# Autodesk Inventor assembly: 021-DXP(F,D-770)
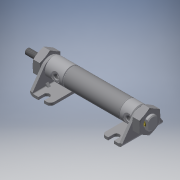
[picture p0: Inventor's stored thumbnail of the model, 180x180]
Saved by Autodesk Inventor 2018 (Build 220112000, 112)
## iProperties
Category: PARTsolutions
Company: BIMBA
Created: 2019-01-18
Part Number: 021-DXP(F,D-770)
Catalog Web Link: www.cadenas.de
Description: Original Line Standard Air Cylinders-Standard Air Cylinders
Vendor: BIMBA
Document SubType Name: Assembly
Designer: psadmin
Manufacturer: BIMBA
PSOL_IDENT_0: {$CADENAS_DATA\23d-libs\bimba\bimba\bimba_imperial\bimba_full_line\original_line_cylinders\standard_
PSOL_IDENT_1: air_cylinders\standard_air_cylinder_asmtab.prj},331 {VTYP=3D},{STYP=ASSTAB},{NB=021-DXP(F,D-770)},{L
PSOL_IDENT_2: INA=021-DXP},{NN=Original Line Standard Air Cylinders},{DATE=21.03.2018 14:31:21},{GEOMDATE=19.03.20
PSOL_IDENT_3: 18 11:39:15},{VERSION=},{LINEID=40},{WBVAR=STROKE,ACTING,MNT,DER,NR,BM,CO,OO,VO,M,EE,EEL,K,Q,Y,G,T,H
PSOL_IDENT_4: L,B,H,SER,SR,NT,W,STPT1,STPT2,STPT3,STPT4,MB,PB,PRC,TB,MN},{WBNUMERIC=STROKE,EEL}  {NB=021-DXP(F,D-7
PSOL_IDENT_5: 70)},{LINA=021-DXP},{KT=DUMMY},{PN=021-DXP},{PNC=021-DXP(F,D-770)},{PNA=(D-770)},{DASH=-},{BORE1=0.5
PSOL_IDENT_6: 6250000},{BORE=9/16\" (02)},{BOREPN=02},{STROKE=1.000},{STROKEALG=[0.011:50/0.001]},{STROKE1=1.000},
PSOL_IDENT_7: {ACTING=D},{ACTINGALG= '' , 'Single Acting (SA)' , 'R' , 'Reverse Single Acting (SA)' , 'D' , 'Doubl
PSOL_IDENT_8: e Acting (SA)' },{ACTINGPN=D},{MNT=XP},{MNTALG= '' , 'Front Nose Mounting (SA)' , 'XP' , 'Double End
PSOL_IDENT_9: or Rear Pivot Mounting (SA)' , 'X' , 'Double End Mounting (SA)' },{TYPE=},{MNTPN=XP},{DER=},{DERALG=
PSOL_IDENT_10: '' , 'N/A' },{NR=},{NRALG= '' , 'N/A' },{NRPN=},{BM=},{BMALG= '' , 'N/A' },{BMPN=},{CO=},{COALG= ''
PSOL_IDENT_11: , 'N/A' },{OO=},{OOALG= '', 'N/A' },{OOPN=},{VO=Z},{VOALG= 'Z' , 'N/A' },{VOPN=},{OOVOPN=},{M=},{MA
PSOL_IDENT_12: LG= '', 'Without Magnet', 'M', 'With Magnet' },{EE=},{EEL=0.000},{EEMAX=49.0000},{EEALG= '', 'Withou
PSOL_IDENT_13: t Extra Extension', 'EE', 'With Extra Extension' },{EELALG=0},{EEPN=},{EEPN1=0.000},{K=},{KALG= '', '
PSOL_IDENT_14: Standard' , 'K' , 'Ports Rotated 90deg K' },{KPN=},{Q=},{QALG= '' , 'N/A' },{QPN=},{Y=},{YALG= '' , '
PSOL_IDENT_15: With Pivot Bushing' },{YPN=},{YCON=Y},{F=},{FALG= '', 'Non-Coated (Standard)', 'F', 'Molycoated' },{
PSOL_IDENT_16: FPN=},{G=},{GPN=},{GPN99=},{T=},{TALG= '' , 'Standard -20° to 200°F (-29° to 95°C)' , 'N' , 'Low Tem
PSOL_IDENT_17: perature' , 'V' , 'High Temperature' },{NPN=},{VPN=},{HL=},{HLALG= '' , 'Without Low Pressure Hydrau
PSOL_IDENT_18: lic' , 'HL' , 'With Low Pressure Hydraulic' },{B=},{BALG= '', 'W/out Bumpers' , 'B' , 'W/ Bumpers' }
PSOL_IDENT_19: ,{BPN=},{H=},{HALG= '', 'N/A' },{HPN=},{SER=},{SERALG= '' , 'Without Spring Extend/Return' , 'JS' , '
PSOL_IDENT_20: With Spring Return' , 'JR' , 'With Spring Extend' },{SR=},{SRALG= '' , 'Standard Stainless Steel' },
PSOL_IDENT_21: {SRPN=},{SRCON=0},{NT=},{NTPN=},{W=},{WALG= '' , 'Without Wiper' , 'W' , 'With Wiper' },{WPN=},{E=},
PSOL_IDENT_22: {EALG= '' , 'Standard Seals/Lube' , 'E' , 'Non-Lube Seals/Lube' },{EPN=},{ST=},{STALG= '' , 'N/A' },
PSOL_IDENT_23: {STPT1=},{STPT1ALG= '' , 'N/A' },{STPT2=},{STPT2ALG= '' , 'N/A' },{STPT3=},{STPT3ALG= '' , 'N/A' },{
PSOL_IDENT_24: STPT4=},{STPT4ALG= '' , 'N/A' },{STPN=},{MB=F,D-770},{MBALG= '' , 'Without Mounting Bracket' , 'F,D-
PSOL_IDENT_25: 770' , 'D-770 (front)'  , 'R,D-770' , 'D-770 (rear)' , '2x,D-770' , 'D-770 (front & rear)'},{MBPN=(F
PSOL_IDENT_26: ,D-770)},{MBPNALL=D-770},{MBPNALLREAR=D-770},{PB=},{PBALG= '' , 'Without Pivot Bracket' , 'D-12321-A'
PSOL_IDENT_27: , 'D-12321-A' },{PBPN=},{PBPNALL=D-12321-A},{PRC=},{PRCALG= '' , 'W/out Pivot Rod Clevis' , 'F,D-85
PSOL_IDENT_28: 0' , 'D-850 (front)' },{PRCPN=},{PRCPNALL=D-850},{TB=},{TBALG= '' , 'N/A' },{TBPN=},{TBPNALL=},{MN=}
PSOL_IDENT_29: ,{MNALG= '' , 'N/A' },{MNPN=},{MNCONF=},{MNCONR=},{TLEN=1.8870},{FRAC=3.5600},{RGCON=},{RGDACCON=R},
PSOL_IDENT_30: {RHCON=P},{RHCON1=P},{RHCONON=1},{RHACCON=R},{FNUTCON=1},{RNUTCON=1},{FNUTPN=D-154},{RNUTPN=D-154},{
PSOL_IDENT_31: FNUTTRANS=0.0000},{RNUTTRANS=0.0000},{VHOLECON=0},{A1=1.1560},{A1N=1.0310},{A1P=1.1560},{A1B=0.0000}
PSOL_IDENT_32: ,{A4=0.1570},{A4N=0.5310},{A4P=0.1570},{A5=0.0250},{A1H=0.969},{A1NH=0.5000},{A1PH=0.9690},{A1BH=0.0
PSOL_IDENT_33: 000},{A1SH=0.0000},{A2H=0.1570},{A2NH=0.1570},{LENGTH=2.5600},{LENGTH1=2.5600},{LENGTH2=2.6100},{MUL=
PSOL_IDENT_34: 1.0000},{MUL11=1.0000},{MUL22=2.63},{MUL33=1.6300},{MUL2=1.0000},{MUL211=1.0000},{MUL222=2.6300},{MU
PSOL_IDENT_35: L233=1.6300},{SSS=2.0000},{RGLEN=1.0240},{RHLEN=0.6490},{SSS1=2.0000},{A13=0.7810},{DIF=0.0000},{G5=
PSOL_IDENT_36: 0.0000},{ON=0},{SSADD=0.0000},{BADD=0.0000},{MADD=0.0000},{NVADD=0.0000},{TRACKL=1.5870},{TRACKCON=D
PSOL_IDENT_37: -74168},{TRIMCON=0},{TRIMCON1=0},{PINCON=},{FSPACE=0.4944},{SPACE=0.0402},{TEXT=0.0703},{S1=0.0000},
PSOL_IDENT_38: {D1=0.0000},{D1N=0.6150},{D1B=0.6150},{D1P=0.0000},{FA=0.690},{RA=0.6900},{PPATH=standard_air_cylind
PSOL_IDENT_39: er_asmtpl.prj},{MATALGHTML=<b>Standard Original Line:</b><dl><dt>Rod:</dt><dd>- Stainless Steel</dd>
PSOL_IDENT_40: <dd>&nbsp;&nbsp;(5/16 9/16 Bores)</dd><dd>- High Strength Carbon Steel</dd><dd>&nbsp;&nbsp;(3/4 3 Bo
PSOL_IDENT_41: re)</dd><dd>- Stainless Steel</dd><dd>&nbsp;&nbsp;(X style DXP/DX/DXDE)</dd><dt>Bearings:</dt><dd>-
PSOL_IDENT_42: Sintered Bronze</dd><dt>Body:</dt><dd>- 304 Stainless Steel</dd><dt>End Caps:</dt><dd>- Aluminum</dd
PSOL_IDENT_43: ><dt>Seals:</dt><dd>- Buna N</dd></dl>},{ASSCFGPRA=02DXP},{MBPNA=(D-770)},{MNPNA=},{PRCPNA=},{ASSOPT
PSOL_IDENT_44: ACC=STPT4},{A=3.56},{HADD=0.0000},{WFL=0},{QADD=0.000},{QADD1=0.030},{TEST=1.0000},{MNTB=},{STDNUTF=
PSOL_IDENT_45: 1},{STDNUTR=1},{STRK2D=0},{X2D=2},{STROKESW=1.000},{EESW=0.000},{FCD=0},{BCD=0},{RCD=0},{CUSTADD=0.0
PSOL_IDENT_46: 00},{FT=#10-32 UNF-2A},{FT1=#10-32 UNF-2A},{FT2=7/16-20 UNF-2A},{PORT=#10-32},{FT11=7/16-20 UNF-2A},
PSOL_IDENT_47: {FT12=7/16-20 UNF-2A},{B1=}
NN: Original Line Standard Air Cylinders
NT: Standard Male Thread
NB: 021-DXP(F,D-770)
NBSYN: $PNC.
LINA: 021-DXP
PN: 021-DXP
PNA: (D-770)
BORE: 9/16" (02)
STROKE: 1
ACTING: Double [D]
MNT: Universal Double End or Rear Pivot [XP]
DER: N/A
NR: N/A
BM: N/A
CO: N/A
OO: N/A
VO: N/A
M: Without Magnet Piston
EE: Standard Rod Extension
EEL: 0
K: Standard
Q: N/A
Y: Pivot Bushing [Y]
G: Standard Grease Lube
T: Standard -20° to 200°F (-29° to 95°C)
HL: Standard 250 PSI Air
B: Without Bumpers
H: N/A
SER: Without Failsafe Spring Extend/Return
SR: Standard Stainless Steel
W: Without Wiper
STPT1: N/A
STPT2: N/A
STPT3: N/A
STPT4: N/A
MB: D-770 (front)
PB: Without Pivot Bracket
PRC: Without Piston Rod Clevis
TB: N/A
MN: N/A
A: 3.56
SUPPLIER: BIMBA
ARTICLENO: 021-DXP(F,D-770)
BOMINFO: 021-DXP
CREATOR: CADENAS GmbH
Title: 021-DXP
Author: Cadenas PARTsolutions
Comments: Standard Air Cylinders
## Documents named in this file (9)
- C:\Users\Burni\Desktop\Robotics\hatch\PARTserver02019011803125824465437192d056f\AIS2018\021-DXP(F,D-770).iam
- C:\Users\Burni\Desktop\Robotics\hatch\PARTserver02019011803125824465437192d056f\AIS2018\021-DXP(F,D-770)0000000_0_dummy.ipt
- C:\Users\Burni\Desktop\Robotics\hatch\PARTserver02019011803125824465437192d056f\AIS2018\02R010-0_rod_guide.ipt
- C:\Users\Burni\Desktop\Robotics\hatch\PARTserver02019011803125824465437192d056f\AIS2018\02R-1_8870.ipt
- C:\Users\Burni\Desktop\Robotics\hatch\PARTserver02019011803125824465437192d056f\AIS2018\02P0Y000_rear_head.ipt
- C:\Users\Burni\Desktop\Robotics\hatch\PARTserver02019011803125824465437192d056f\AIS2018\D-154.ipt
- C:\Users\Burni\Desktop\Robotics\hatch\PARTserver02019011803125824465437192d056f\AIS2018\D-8597.ipt
- C:\Users\Burni\Desktop\Robotics\hatch\PARTserver02019011803125824465437192d056f\AIS2018\D-770.ipt
- C:\Users\Burni\Desktop\Robotics\hatch\PARTserver02019011803125824465437192d056f\AIS2018\021-DXP0000_rod.ipt
## Components (10 placed, 8 different names)
1. 021-DXP(F,D-770)0000000_0_dummy:1
2. 02R010-0_rod_guide:1
3. 02R-1_8870:1
4. 02P0Y000_rear_head:1 — Mate:1, Mate:2, Mate:4
5. D-8597:1
6. D-154:2
7. D-770:1 — Flush:1
8. 021-DXP0000_rod:1
9. D-770:2 — Mate:1, Flush:1, Mate:2, Mate:3
10. D-154:3 — Mate:3, Mate:4
## Relationships (5: Mate 4, Flush 1)
- Mate:1: 02P0Y000_rear_head:1 ↔ D-770:2
- Flush:1: D-770:1 ↔ D-770:2
- Mate:2: 02P0Y000_rear_head:1 ↔ D-770:2
- Mate:3: D-770:2 ↔ D-154:3
- Mate:4: 02P0Y000_rear_head:1 ↔ D-154:3
